# Autodesk Inventor assembly: left_femalejoint
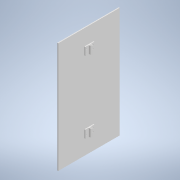
[picture p0: Inventor's stored thumbnail of the model, 180x180]
Saved by Autodesk Inventor 2020 (Build 240168000, 168)
## iProperties
Created: 2020-05-03
Part Number: left_femalejoint
Document SubType Name: Assembly
Designer: galaxy
Author: galaxy
## Documents named in this file (3)
- C:\Users\galaxy\Desktop\control box\left_femalejoint.iam
- C:\Users\galaxy\Desktop\control box\leftside.ipt
- C:\Users\galaxy\Desktop\control box\joint_female.ipt
## Components (3 placed, 2 different names)
1. leftside:1 — Insert:1, Insert:2, Insert:3, Insert:4
2. joint_female:1 — Insert:1, Insert:2
3. joint_female:2 — Insert:3, Insert:4
## Relationships (4: Insert 4)
- Insert:1: leftside:1 ↔ joint_female:1
- Insert:2: leftside:1 ↔ joint_female:1
- Insert:3: leftside:1 ↔ joint_female:2
- Insert:4: leftside:1 ↔ joint_female:2
